# Autodesk Inventor assembly: Cube 1x1 V5 Alt
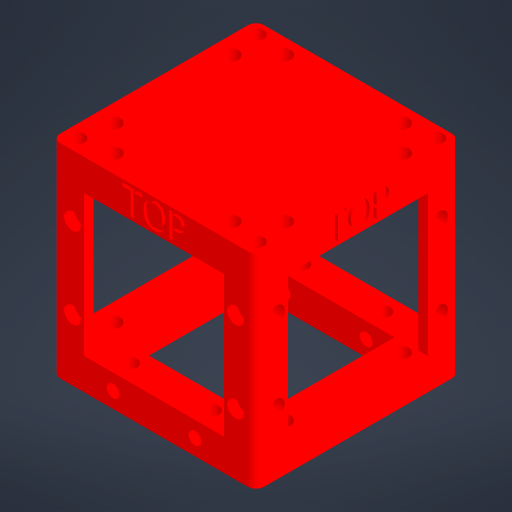
[picture p0: Inventor's stored thumbnail of the model, 512x512]
Saved by Autodesk Inventor 2023.4 (Build 274418000, 418)
## iProperties
Created: 2024-05-07
Part Number: Cube 1x1 V5 Alt
Document SubType Name: Assembly
Designer: xSibe
Author: xSibe
## Documents named in this file (3)
- C:\.Laptop\.Work\Projects\Project Protocube\1 Autodesk\1 Cubes\Cubes\Cube 1x1 V5 Alt.iam
- C:\.Laptop\.Work\Projects\Project Protocube\1 Autodesk\1 Cubes\Cubes\Cube 1x1 Bottom V5.ipt
- C:\.Laptop\.Work\Projects\Project Protocube\1 Autodesk\1 Cubes\Cubes\Cube 1x1 Top V5 Closed.ipt
## Components (2 placed, 2 different names)
1. Cube 1x1 Bottom V5:1 — Mate:1, Mate:2, Mate:3
2. Cube 1x1 Top V5 Closed:1 — Mate:1, Mate:2, Mate:3
## Relationships (3: Mate 3)
- Mate:1: Cube 1x1 Bottom V5:1 ↔ Cube 1x1 Top V5 Closed:1
- Mate:2: Cube 1x1 Bottom V5:1 ↔ Cube 1x1 Top V5 Closed:1
- Mate:3: Cube 1x1 Bottom V5:1 ↔ Cube 1x1 Top V5 Closed:1
